# Autodesk Inventor assembly: DriveTrainPlate
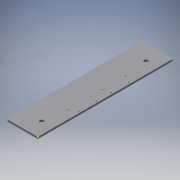
[picture p0: Inventor's stored thumbnail of the model, 180x180]
Saved by Autodesk Inventor 2016 (Build 200138000, 138)
## iProperties
Created: 2016-09-21
Part Number: DriveTrainPlate
Document SubType Name: Assembly
Designer: RoboticsUser
Author: RoboticsUser
## Documents named in this file (3)
- C:\Robotics\2016-17_CAD\DriveTrainPlate.iam
- C:\Robotics\2016-17_CAD\DriveTrainPlate.ipt
- C:\Users\RoboticsUser\Desktop\2015-16 CAD\COTSParts\Actobotics\585 parts\585450.ipt
## Components (2 placed, 2 different names)
1. DriveTrainPlate:1 — Mate:1, Flush:1, Flush:2
2. 585450:1 — Mate:1, Flush:1, Flush:2
## Relationships (3: Flush 2, Mate 1)
- Mate:1: DriveTrainPlate:1 ↔ 585450:1
- Flush:1 (107.95 mm): DriveTrainPlate:1 ↔ 585450:1
- Flush:2: DriveTrainPlate:1 ↔ 585450:1
